# Autodesk Inventor assembly: 2024-210-Fixed-Shootaur
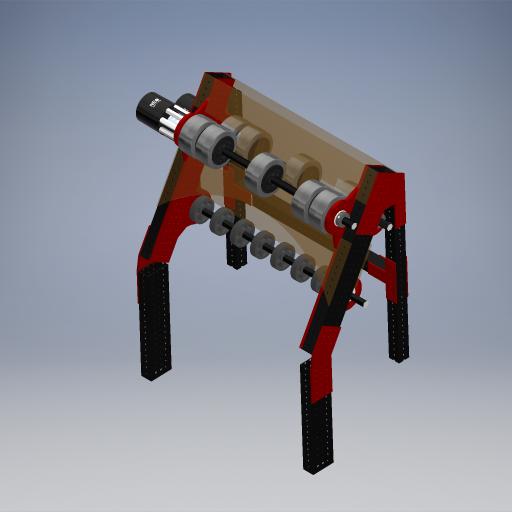
[picture p0: Inventor's stored thumbnail of the model, 512x512]
Saved by Autodesk Inventor 2024.2 (Build 282272000, 272)
## iProperties
Created: 2024-02-11
Part Number: 2024-210-Fixed-Shootaur
Document SubType Name: Assembly
Designer: rohan
Author: rohan
## Documents named in this file (23)
- C:\Users\rohan\OneDrive - Hillsborough County Public Schools\Robotics\FIRST-Robotics-Competition\Crescendo\Minotaur-Crescendo-Robot\Structure\Superstructure\Fixed Shooter\2024-210-Fixed-Shootaur.iam
- C:\Users\rohan\OneDrive - Hillsborough County Public Schools\Robotics\FIRST-Robotics-Competition\Crescendo\Minotaur-Crescendo-Robot\Structure\Superstructure\Fixed Shooter\2024-210-004-Back-Gusset.ipt
- C:\Users\rohan\OneDrive - Hillsborough County Public Schools\Robotics\FIRST-Robotics-Competition\Crescendo\Minotaur-Crescendo-Robot\Structure\Superstructure\Fixed Shooter\2024-210-005-Front-Gusset.ipt
- C:\Users\rohan\OneDrive - Hillsborough County Public Schools\Robotics\FIRST-Robotics-Competition\Crescendo\Minotaur-Crescendo-Robot\Structure\Superstructure\Fixed Shooter\2024-210-001-Shooter-Beam.ipt
- C:\Users\rohan\OneDrive - Hillsborough County Public Schools\Robotics\FIRST-Robotics-Competition\Crescendo\Minotaur-Crescendo-Robot\Structure\Superstructure\Fixed Shooter\2024-210-003-Front-Angle.ipt
- C:\Users\rohan\OneDrive - Hillsborough County Public Schools\Robotics\FIRST-Robotics-Competition\Crescendo\Minotaur-Crescendo-Robot\Structure\Superstructure\Fixed Shooter\2024-210-002-Backright-Support.ipt
- C:\Users\rohan\OneDrive - Hillsborough County Public Schools\Robotics\FIRST-Robotics-Competition\Crescendo\Minotaur-Crescendo-Robot\Structure\Superstructure\Fixed Shooter\2024-210-007-Left-Right-Support.ipt
- C:\Users\rohan\OneDrive - Hillsborough County Public Schools\Robotics\FIRST-Robotics-Competition\Crescendo\Minotaur-Crescendo-Robot\Structure\Gussets\THRIFYBOT-T-Gusset.ipt
- C:\Users\rohan\OneDrive - Hillsborough County Public Schools\Robotics\FIRST-Robotics-Competition\Crescendo\Minotaur-Crescendo-Robot\Structure\Superstructure\Polycarbonate-Note-Intakaur-Cover - Copy.ipt
- C:\Users\rohan\OneDrive - Hillsborough County Public Schools\Robotics\FIRST-Robotics-Competition\Crescendo\Minotaur-Crescendo-Robot\Structure\Superstructure\Fixed Shooter\2024-210-009-Shooter-Gusset-Plate.ipt
- C:\Users\rohan\OneDrive - Hillsborough County Public Schools\Robotics\FIRST-Robotics-Competition\Crescendo\Minotaur-Crescendo-Robot\Electronics\Neo-Brushless-Motors\NEO-Brushless-Motor-V1.1.ipt
- C:\Users\rohan\OneDrive - Hillsborough County Public Schools\Robotics\FIRST-Robotics-Competition\Crescendo\Minotaur-Crescendo-Robot\Motion\Adapters\0.5-inch-Hex-Shaft-Coupler.ipt
- C:\Users\rohan\OneDrive - Hillsborough County Public Schools\Robotics\FIRST-Robotics-Competition\Crescendo\Minotaur-Crescendo-Robot\Motion\Adapters\8mm-to-HEX.ipt
- C:\Users\rohan\OneDrive - Hillsborough County Public Schools\Robotics\FIRST-Robotics-Competition\Crescendo\Minotaur-Crescendo-Robot\Motion\Shafting\2024-210-010-Shooter-HEX-Shaft.ipt
- C:\Users\rohan\OneDrive - Hillsborough County Public Schools\Robotics\FIRST-Robotics-Competition\Crescendo\Minotaur-Crescendo-Robot\Motion\Wheels\3in-Colson-Performa.ipt
- C:\Users\rohan\OneDrive - Hillsborough County Public Schools\Robotics\FIRST-Robotics-Competition\Crescendo\Minotaur-Crescendo-Robot\Motion\Bearings\HEX-Bearing (1.125in OD).ipt
- C:\Users\rohan\OneDrive - Hillsborough County Public Schools\Robotics\FIRST-Robotics-Competition\Crescendo\Minotaur-Crescendo-Robot\Motion\Shafting\2024-210-011-Dead-Note-Guide.ipt
- C:\Users\rohan\OneDrive - Hillsborough County Public Schools\Robotics\FIRST-Robotics-Competition\Crescendo\Minotaur-Crescendo-Robot\Motion\Adapters\0.5-inch-HEX-Shaft-Collar (High Strength, Balanced).ipt
- C:\Users\rohan\OneDrive - Hillsborough County Public Schools\Robotics\FIRST-Robotics-Competition\Crescendo\Minotaur-Crescendo-Robot\Structure\Standoffs\Spacers__Standoffs.ipt
- C:\Users\rohan\OneDrive - Hillsborough County Public Schools\Robotics\FIRST-Robotics-Competition\Crescendo\Minotaur-Crescendo-Robot\Structure\Standoffs\Spacers__Standoffs\Aluminum Hex Standoff (No. 10x32 x 1.5Lg x 0.375OD).ipt
- C:\Users\rohan\OneDrive - Hillsborough County Public Schools\Robotics\FIRST-Robotics-Competition\Crescendo\Minotaur-Crescendo-Robot\Structure\Standoffs\Spacers__Standoffs\Aluminum Hex Standoff (No. 10x32 x 1.75Lg x 0.375OD).ipt
- C:\Users\rohan\OneDrive - Hillsborough County Public Schools\Robotics\FIRST-Robotics-Competition\Crescendo\Minotaur-Crescendo-Robot\Structure\Superstructure\Polycarbonate-Bottom-Shooter-Rest.ipt
- C:\Users\rohan\OneDrive - Hillsborough County Public Schools\Robotics\FIRST-Robotics-Competition\Crescendo\Minotaur-Crescendo-Robot\Motion\Wheels\2in-Compliant-Wheels-45A.ipt
## Components (63 placed, 21 different names)
1. 2024-210-004-Back-Gusset:1 — Flush:9, Mate:44, Flush:55, Flush:60
2. 2024-210-005-Front-Gusset:2 — Flush:23, Mate:22, Flush:24, Mate:25, Flush:26, Mate:26
3. 2024-210-001-Shooter-Beam:1 — Flush:23, Mate:22, Flush:24, Mate:38, Flush:48, Flush:49, Flush:52, Mate:40, Flush:53, Mate:44, Flush:55, Mate:169, Flush:57, Flush:58, Flush:60
4. 2024-210-002-Backright-Support:1 — Flush:9, Flush:19, Flush:20, Mate:13
5. 2024-210-004-Back-Gusset:4 — Flush:59
6. 2024-210-005-Front-Gusset:3 — Mate:21, Flush:21, Flush:22, Mate:23, Flush:25, Mate:24
7. 2024-210-001-Shooter-Beam:2 — Mate:21, Flush:21, Flush:22, Mate:39, Flush:50, Flush:51, Insert:8, Flush:59
8. 2024-210-002-Backright-Support:2 — Flush:19, Flush:20, Mate:13
9. 2024-210-003-Front-Angle:1 — Mate:25, Flush:26, Mate:26, Mate:28, Mate:36, Flush:44, Flush:54
10. 2024-210-003-Front-Angle:2 — Mate:23, Flush:25, Mate:24, Flush:29, Mate:35, Flush:43, Insert:7, Flush:54
11. 2024-210-007-Left-Right-Support:1 — Mate:28, Flush:29, Flush:42, Flush:45, Mate:43
12. THRIFYBOT-T-Gusset:1 — Flush:38, Flush:39, Mate:33, Mate:35, Flush:42, Flush:43, Insert:7
13. THRIFYBOT-T-Gusset:2 — Flush:38, Flush:39, Mate:33
14. THRIFYBOT-T-Gusset:3 — Mate:36, Flush:44, Flush:45
15. THRIFYBOT-T-Gusset:4 — Mate:43
16. Polycarbonate-Note-Intakaur-Cover - Copy:1 — Mate:38, Flush:48, Flush:49, Insert:8
17. 2024-210-009-Shooter-Gusset-Plate:1 — Mate:39, Flush:50, Flush:51, Symmetry:1, Mate:137, Mate:138, Mate:157, Mate:158, Mate:159, Mate:160
18. 2024-210-009-Shooter-Gusset-Plate:2 — Flush:52, Mate:40, Flush:53, Mate:58, Mate:59, Mate:67, Mate:68, Mate:95, Mate:103, Symmetry:1, Mate:135, Mate:136, Mate:147, Mate:148, Mate:150, Mate:151, Mate:152, Mate:153, Mate:155, Mate:156, Mate:161, Mate:162
19. NEO-Brushless-Motor-V1.1:1 — Mate:58, Mate:59, Mate:102, Mate:123, Mate:149
20. NEO-Brushless-Motor-V1.1:2 — Mate:67, Mate:68, Mate:94, Mate:122, Mate:154
21. 0.5-inch-Hex-Shaft-Coupler:1 — Mate:88, Mate:89, Mate:90, Mate:91, Mate:95, Mate:122
22. 8mm-to-HEX:1 — Mate:88, Mate:89, Mate:92, Mate:93, Mate:94
23. 2024-210-010-Shooter-HEX-Shaft:1 — Mate:90, Mate:91, Mate:92, Mate:116, Mate:117, Mate:118, Mate:119, Mate:124, Mate:125, Mate:126, Mate:127, Mate:131, Mate:132, Mate:163, Mate:164
24. 0.5-inch-Hex-Shaft-Coupler:5 — Mate:103, Mate:123
25. 8mm-to-HEX:5 — Mate:101, Mate:102
26. 2024-210-010-Shooter-HEX-Shaft:2 — Mate:104, Mate:105, Mate:106, Mate:107, Mate:110, Mate:111, Mate:112, Mate:113, Mate:129, Mate:130, Mate:166, Mate:167
27. 3in-Colson-Performa:1 — Mate:124, Mate:125, Mate:128, Mate:191
28. 3in-Colson-Performa:2 — Mate:110, Mate:111, Mate:114, Mate:189
29. 3in-Colson-Performa:3 — Mate:106, Mate:107, Mate:109, Mate:133
30. 3in-Colson-Performa:4 — Mate:104, Mate:105, Mate:109, Mate:192
31. 3in-Colson-Performa:5 — Mate:112, Mate:113, Mate:114
32. 3in-Colson-Performa:6 — Mate:116, Mate:117, Mate:120, Mate:190
33. 3in-Colson-Performa:7 — Mate:118, Mate:119, Mate:120
34. 3in-Colson-Performa:8 — Mate:126, Mate:127, Mate:128, Mate:134
35. 3in-Colson-Performa:9 — Mate:129, Mate:130, Mate:133
36. 3in-Colson-Performa:10 — Mate:131, Mate:132, Mate:134
37. HEX-Bearing (1.125in OD):1 — Mate:137, Mate:138, Mate:139, Mate:140
38. HEX-Bearing (1.125in OD):2 — Mate:135, Mate:136, Mate:188, Insert:9
39. 2024-210-011-Dead-Note-Guide:1 — Mate:139, Mate:140, Mate:188
40. Aluminum Hex Standoff (No. 10x32 x 1.5Lg x 0.375OD):6 — Mate:152, Mate:153
41. HEX-Bearing (1.125in OD):3 — Mate:155, Mate:156, Mate:192
42. HEX-Bearing (1.125in OD):4 — Mate:157, Mate:158, Mate:168, Mate:189
43. HEX-Bearing (1.125in OD):5 — Mate:161, Mate:162, Mate:191
44. HEX-Bearing (1.125in OD):6 — Mate:159, Mate:160, Mate:165, Mate:190
45. 0.5-inch-HEX-Shaft-Collar (High Strength, Balanced):5 — Mate:163, Mate:164, Mate:165
46. 0.5-inch-HEX-Shaft-Collar (High Strength, Balanced):7 — Mate:166, Mate:167, Mate:168
47. Polycarbonate-Bottom-Shooter-Rest:1 — Mate:169, Flush:57, Flush:58
48. Aluminum Hex Standoff (No. 10x32 x 1.75Lg x 0.375OD):1 — Mate:147, Mate:148
49. Aluminum Hex Standoff (No. 10x32 x 1.75Lg x 0.375OD):7
50. Aluminum Hex Standoff (No. 10x32 x 1.75Lg x 0.375OD):8
51. Aluminum Hex Standoff (No. 10x32 x 1.75Lg x 0.375OD):9
52. Aluminum Hex Standoff (No. 10x32 x 1.75Lg x 0.375OD):10
53. Aluminum Hex Standoff (No. 10x32 x 1.75Lg x 0.375OD):11 — Mate:149
54. Aluminum Hex Standoff (No. 10x32 x 1.75Lg x 0.375OD):4 — Mate:150, Mate:151
55. Aluminum Hex Standoff (No. 10x32 x 1.75Lg x 0.375OD):12 — Mate:154
56. 2in-Compliant-Wheels-45A:8 — Insert:9
57. 2in-Compliant-Wheels-45A:9
58. 2in-Compliant-Wheels-45A:10
59. 2in-Compliant-Wheels-45A:11
60. 2in-Compliant-Wheels-45A:12
61. 2in-Compliant-Wheels-45A:13
62. 2in-Compliant-Wheels-45A:14
63. 2in-Compliant-Wheels-45A:15
## Component patterns: (6 elements, first: Aluminum Hex Standoff (No. 10x32 x 1.75Lg x 0.375OD):1), (2 elements, first: Aluminum Hex Standoff (No. 10x32 x 1.75Lg x 0.375OD):4), (8 elements, first: 2in-Compliant-Wheels-45A:8)
## Relationships (138: Mate 101, Flush 31, Insert 5, Symmetry 1)
- Flush:9: 2024-210-004-Back-Gusset:1 ↔ 2024-210-002-Backright-Support:1
- [Mate]: 2024-210-004-Back-Gusset:4 ↔ 2024-210-001-Shooter-Beam:2
- [Flush]: 2024-210-004-Back-Gusset:4 ↔ 2024-210-001-Shooter-Beam:2
- [Insert]: 2024-210-004-Back-Gusset:4 ↔ 2024-210-001-Shooter-Beam:2
- [Mate]: 2024-210-004-Back-Gusset:4 ↔ 2024-210-002-Backright-Support:2
- [Insert]: 2024-210-004-Back-Gusset:4 ↔ 2024-210-002-Backright-Support:2
- Flush:19: 2024-210-002-Backright-Support:1 ↔ 2024-210-002-Backright-Support:2
- Flush:20: 2024-210-002-Backright-Support:1 ↔ 2024-210-002-Backright-Support:2
- Mate:13 (381 mm): 2024-210-002-Backright-Support:1 ↔ 2024-210-002-Backright-Support:2
- Mate:21: 2024-210-005-Front-Gusset:3 ↔ 2024-210-001-Shooter-Beam:2
- Flush:21: 2024-210-005-Front-Gusset:3 ↔ 2024-210-001-Shooter-Beam:2
- Flush:22: 2024-210-005-Front-Gusset:3 ↔ 2024-210-001-Shooter-Beam:2
- Flush:23: 2024-210-005-Front-Gusset:2 ↔ 2024-210-001-Shooter-Beam:1
- Mate:22: 2024-210-005-Front-Gusset:2 ↔ 2024-210-001-Shooter-Beam:1
- Flush:24: 2024-210-005-Front-Gusset:2 ↔ 2024-210-001-Shooter-Beam:1
- Mate:23: 2024-210-005-Front-Gusset:3 ↔ 2024-210-003-Front-Angle:2
- Flush:25: 2024-210-005-Front-Gusset:3 ↔ 2024-210-003-Front-Angle:2
- Mate:24: 2024-210-005-Front-Gusset:3 ↔ 2024-210-003-Front-Angle:2
- Mate:25: 2024-210-005-Front-Gusset:2 ↔ 2024-210-003-Front-Angle:1
- Flush:26: 2024-210-005-Front-Gusset:2 ↔ 2024-210-003-Front-Angle:1
- Mate:26: 2024-210-005-Front-Gusset:2 ↔ 2024-210-003-Front-Angle:1
- Mate:28: 2024-210-003-Front-Angle:1 ↔ 2024-210-007-Left-Right-Support:1
- Flush:29: 2024-210-003-Front-Angle:2 ↔ 2024-210-007-Left-Right-Support:1
- Flush:38: THRIFYBOT-T-Gusset:1 ↔ THRIFYBOT-T-Gusset:2
- Flush:39: THRIFYBOT-T-Gusset:1 ↔ THRIFYBOT-T-Gusset:2
- Mate:33 (25.4 mm): THRIFYBOT-T-Gusset:1 ↔ THRIFYBOT-T-Gusset:2
- [Flush]: THRIFYBOT-T-Gusset:3 ↔ THRIFYBOT-T-Gusset:4
- [Flush]: THRIFYBOT-T-Gusset:3 ↔ THRIFYBOT-T-Gusset:4
- [Mate] (25.4 mm): THRIFYBOT-T-Gusset:3 ↔ THRIFYBOT-T-Gusset:4
- Mate:35: 2024-210-003-Front-Angle:2 ↔ THRIFYBOT-T-Gusset:1
- Flush:42: 2024-210-007-Left-Right-Support:1 ↔ THRIFYBOT-T-Gusset:1
- Flush:43: 2024-210-003-Front-Angle:2 ↔ THRIFYBOT-T-Gusset:1
- Mate:36: 2024-210-003-Front-Angle:1 ↔ THRIFYBOT-T-Gusset:3
- Flush:44: 2024-210-003-Front-Angle:1 ↔ THRIFYBOT-T-Gusset:3
- Flush:45: 2024-210-007-Left-Right-Support:1 ↔ THRIFYBOT-T-Gusset:3
- Mate:38: 2024-210-001-Shooter-Beam:1 ↔ Polycarbonate-Note-Intakaur-Cover - Copy:1
- Flush:48: 2024-210-001-Shooter-Beam:1 ↔ Polycarbonate-Note-Intakaur-Cover - Copy:1
- Flush:49: 2024-210-001-Shooter-Beam:1 ↔ Polycarbonate-Note-Intakaur-Cover - Copy:1
- Insert:7: 2024-210-003-Front-Angle:2 ↔ THRIFYBOT-T-Gusset:1
- Mate:39: 2024-210-001-Shooter-Beam:2 ↔ 2024-210-009-Shooter-Gusset-Plate:1
- Flush:50: 2024-210-001-Shooter-Beam:2 ↔ 2024-210-009-Shooter-Gusset-Plate:1
- Flush:51: 2024-210-001-Shooter-Beam:2 ↔ 2024-210-009-Shooter-Gusset-Plate:1
- Flush:52: 2024-210-001-Shooter-Beam:1 ↔ 2024-210-009-Shooter-Gusset-Plate:2
- Mate:40: 2024-210-001-Shooter-Beam:1 ↔ 2024-210-009-Shooter-Gusset-Plate:2
- Flush:53: 2024-210-001-Shooter-Beam:1 ↔ 2024-210-009-Shooter-Gusset-Plate:2
- Mate:43: 2024-210-007-Left-Right-Support:1 ↔ THRIFYBOT-T-Gusset:4
- Mate:44: 2024-210-004-Back-Gusset:1 ↔ 2024-210-001-Shooter-Beam:1
- Flush:54: 2024-210-003-Front-Angle:1 ↔ 2024-210-003-Front-Angle:2
- Insert:8: 2024-210-001-Shooter-Beam:2 ↔ Polycarbonate-Note-Intakaur-Cover - Copy:1
- Mate:58: 2024-210-009-Shooter-Gusset-Plate:2 ↔ NEO-Brushless-Motor-V1.1:1
- Mate:59: 2024-210-009-Shooter-Gusset-Plate:2 ↔ NEO-Brushless-Motor-V1.1:1
- Mate:67: 2024-210-009-Shooter-Gusset-Plate:2 ↔ NEO-Brushless-Motor-V1.1:2
- Mate:68: 2024-210-009-Shooter-Gusset-Plate:2 ↔ NEO-Brushless-Motor-V1.1:2
- Flush:55: 2024-210-004-Back-Gusset:1 ↔ 2024-210-001-Shooter-Beam:1
- Mate:88: 0.5-inch-Hex-Shaft-Coupler:1 ↔ 8mm-to-HEX:1
- Mate:89: 0.5-inch-Hex-Shaft-Coupler:1 ↔ 8mm-to-HEX:1
- Mate:90: 0.5-inch-Hex-Shaft-Coupler:1 ↔ 2024-210-010-Shooter-HEX-Shaft:1
- Mate:91: 0.5-inch-Hex-Shaft-Coupler:1 ↔ 2024-210-010-Shooter-HEX-Shaft:1
- Mate:92: 8mm-to-HEX:1 ↔ 2024-210-010-Shooter-HEX-Shaft:1
- Mate:93: 8mm-to-HEX:1
- Mate:94: NEO-Brushless-Motor-V1.1:2 ↔ 8mm-to-HEX:1
- Mate:95: 2024-210-009-Shooter-Gusset-Plate:2 ↔ 0.5-inch-Hex-Shaft-Coupler:1
- [Mate]: 0.5-inch-Hex-Shaft-Coupler:5 ↔ 8mm-to-HEX:5
- [Mate]: 0.5-inch-Hex-Shaft-Coupler:5 ↔ 8mm-to-HEX:5
- [Mate]: 0.5-inch-Hex-Shaft-Coupler:5 ↔ 2024-210-010-Shooter-HEX-Shaft:2
- [Mate]: 0.5-inch-Hex-Shaft-Coupler:5 ↔ 2024-210-010-Shooter-HEX-Shaft:2
- [Mate]: 8mm-to-HEX:5 ↔ 2024-210-010-Shooter-HEX-Shaft:2
- Mate:101: 8mm-to-HEX:5
- Mate:102: NEO-Brushless-Motor-V1.1:1 ↔ 8mm-to-HEX:5
- Mate:103: 2024-210-009-Shooter-Gusset-Plate:2 ↔ 0.5-inch-Hex-Shaft-Coupler:5
- Mate:104: 2024-210-010-Shooter-HEX-Shaft:2 ↔ 3in-Colson-Performa:4
- Mate:105: 2024-210-010-Shooter-HEX-Shaft:2 ↔ 3in-Colson-Performa:4
- Mate:106: 2024-210-010-Shooter-HEX-Shaft:2 ↔ 3in-Colson-Performa:3
- Mate:107: 2024-210-010-Shooter-HEX-Shaft:2 ↔ 3in-Colson-Performa:3
- Mate:109: 3in-Colson-Performa:3 ↔ 3in-Colson-Performa:4
- Mate:110: 2024-210-010-Shooter-HEX-Shaft:2 ↔ 3in-Colson-Performa:2
- Mate:111: 2024-210-010-Shooter-HEX-Shaft:2 ↔ 3in-Colson-Performa:2
- Mate:112: 2024-210-010-Shooter-HEX-Shaft:2 ↔ 3in-Colson-Performa:5
- Mate:113: 2024-210-010-Shooter-HEX-Shaft:2 ↔ 3in-Colson-Performa:5
- Mate:114: 3in-Colson-Performa:2 ↔ 3in-Colson-Performa:5
- Mate:116: 2024-210-010-Shooter-HEX-Shaft:1 ↔ 3in-Colson-Performa:6
- Mate:117: 2024-210-010-Shooter-HEX-Shaft:1 ↔ 3in-Colson-Performa:6
- Mate:118: 2024-210-010-Shooter-HEX-Shaft:1 ↔ 3in-Colson-Performa:7
- Mate:119: 2024-210-010-Shooter-HEX-Shaft:1 ↔ 3in-Colson-Performa:7
- Mate:120: 3in-Colson-Performa:6 ↔ 3in-Colson-Performa:7
- Mate:122: NEO-Brushless-Motor-V1.1:2 ↔ 0.5-inch-Hex-Shaft-Coupler:1
- Mate:123: NEO-Brushless-Motor-V1.1:1 ↔ 0.5-inch-Hex-Shaft-Coupler:5
- Mate:124: 2024-210-010-Shooter-HEX-Shaft:1 ↔ 3in-Colson-Performa:1
- Mate:125: 2024-210-010-Shooter-HEX-Shaft:1 ↔ 3in-Colson-Performa:1
- Mate:126: 2024-210-010-Shooter-HEX-Shaft:1 ↔ 3in-Colson-Performa:8
- Mate:127: 2024-210-010-Shooter-HEX-Shaft:1 ↔ 3in-Colson-Performa:8
- Mate:128: 3in-Colson-Performa:1 ↔ 3in-Colson-Performa:8
- Mate:129: 2024-210-010-Shooter-HEX-Shaft:2 ↔ 3in-Colson-Performa:9
- Mate:130: 2024-210-010-Shooter-HEX-Shaft:2 ↔ 3in-Colson-Performa:9
- Mate:131: 2024-210-010-Shooter-HEX-Shaft:1 ↔ 3in-Colson-Performa:10
- Mate:132: 2024-210-010-Shooter-HEX-Shaft:1 ↔ 3in-Colson-Performa:10
- Symmetry:1: 2024-210-009-Shooter-Gusset-Plate:1 ↔ 2024-210-009-Shooter-Gusset-Plate:2
- Mate:133 (81.28 mm): 3in-Colson-Performa:3 ↔ 3in-Colson-Performa:9
- Mate:134 (81.28 mm): 3in-Colson-Performa:8 ↔ 3in-Colson-Performa:10
- Mate:135: 2024-210-009-Shooter-Gusset-Plate:2 ↔ HEX-Bearing (1.125in OD):2
- Mate:136: 2024-210-009-Shooter-Gusset-Plate:2 ↔ HEX-Bearing (1.125in OD):2
- Mate:137: 2024-210-009-Shooter-Gusset-Plate:1 ↔ HEX-Bearing (1.125in OD):1
- Mate:138: 2024-210-009-Shooter-Gusset-Plate:1 ↔ HEX-Bearing (1.125in OD):1
- Mate:139: HEX-Bearing (1.125in OD):1 ↔ 2024-210-011-Dead-Note-Guide:1
- Mate:140: HEX-Bearing (1.125in OD):1 ↔ 2024-210-011-Dead-Note-Guide:1
- Mate:147: 2024-210-009-Shooter-Gusset-Plate:2 ↔ Aluminum Hex Standoff (No. 10x32 x 1.75Lg x 0.375OD):1
- Mate:148: 2024-210-009-Shooter-Gusset-Plate:2 ↔ Aluminum Hex Standoff (No. 10x32 x 1.75Lg x 0.375OD):1
- Mate:149: NEO-Brushless-Motor-V1.1:1 ↔ Aluminum Hex Standoff (No. 10x32 x 1.75Lg x 0.375OD):11
- Mate:150: 2024-210-009-Shooter-Gusset-Plate:2 ↔ Aluminum Hex Standoff (No. 10x32 x 1.75Lg x 0.375OD):4
- Mate:151: 2024-210-009-Shooter-Gusset-Plate:2 ↔ Aluminum Hex Standoff (No. 10x32 x 1.75Lg x 0.375OD):4
- Mate:152: 2024-210-009-Shooter-Gusset-Plate:2 ↔ Aluminum Hex Standoff (No. 10x32 x 1.5Lg x 0.375OD):6
- Mate:153: 2024-210-009-Shooter-Gusset-Plate:2 ↔ Aluminum Hex Standoff (No. 10x32 x 1.5Lg x 0.375OD):6
- Mate:154: NEO-Brushless-Motor-V1.1:2 ↔ Aluminum Hex Standoff (No. 10x32 x 1.75Lg x 0.375OD):12
- Mate:155: 2024-210-009-Shooter-Gusset-Plate:2 ↔ HEX-Bearing (1.125in OD):3
- Mate:156: 2024-210-009-Shooter-Gusset-Plate:2 ↔ HEX-Bearing (1.125in OD):3
- Mate:157: 2024-210-009-Shooter-Gusset-Plate:1 ↔ HEX-Bearing (1.125in OD):4
- Mate:158: 2024-210-009-Shooter-Gusset-Plate:1 ↔ HEX-Bearing (1.125in OD):4
- Mate:159: 2024-210-009-Shooter-Gusset-Plate:1 ↔ HEX-Bearing (1.125in OD):6
- Mate:160: 2024-210-009-Shooter-Gusset-Plate:1 ↔ HEX-Bearing (1.125in OD):6
- Mate:161: 2024-210-009-Shooter-Gusset-Plate:2 ↔ HEX-Bearing (1.125in OD):5
- Mate:162: 2024-210-009-Shooter-Gusset-Plate:2 ↔ HEX-Bearing (1.125in OD):5
- Mate:163: 2024-210-010-Shooter-HEX-Shaft:1 ↔ 0.5-inch-HEX-Shaft-Collar (High Strength, Balanced):5
- Mate:164: 2024-210-010-Shooter-HEX-Shaft:1 ↔ 0.5-inch-HEX-Shaft-Collar (High Strength, Balanced):5
- Mate:165: HEX-Bearing (1.125in OD):6 ↔ 0.5-inch-HEX-Shaft-Collar (High Strength, Balanced):5
- Mate:166: 2024-210-010-Shooter-HEX-Shaft:2 ↔ 0.5-inch-HEX-Shaft-Collar (High Strength, Balanced):7
- Mate:167: 2024-210-010-Shooter-HEX-Shaft:2 ↔ 0.5-inch-HEX-Shaft-Collar (High Strength, Balanced):7
- Mate:168: HEX-Bearing (1.125in OD):4 ↔ 0.5-inch-HEX-Shaft-Collar (High Strength, Balanced):7
- Mate:169: 2024-210-001-Shooter-Beam:1 ↔ Polycarbonate-Bottom-Shooter-Rest:1
- Flush:57: 2024-210-001-Shooter-Beam:1 ↔ Polycarbonate-Bottom-Shooter-Rest:1
- Flush:58: 2024-210-001-Shooter-Beam:1 ↔ Polycarbonate-Bottom-Shooter-Rest:1
- Mate:188: HEX-Bearing (1.125in OD):2 ↔ 2024-210-011-Dead-Note-Guide:1
- Mate:189: 3in-Colson-Performa:2 ↔ HEX-Bearing (1.125in OD):4
- Mate:190: 3in-Colson-Performa:6 ↔ HEX-Bearing (1.125in OD):6
- Mate:191: 3in-Colson-Performa:1 ↔ HEX-Bearing (1.125in OD):5
- Mate:192: 3in-Colson-Performa:4 ↔ HEX-Bearing (1.125in OD):3
- Flush:59: 2024-210-004-Back-Gusset:4 ↔ 2024-210-001-Shooter-Beam:2
- Flush:60: 2024-210-004-Back-Gusset:1 ↔ 2024-210-001-Shooter-Beam:1
- Insert:9 (-13.3096 mm): HEX-Bearing (1.125in OD):2 ↔ 2in-Compliant-Wheels-45A:8
## Named parameters: d24_d6 = 0 mm, d25_d7 = 0 mm, d26_d8 = 0 mm, d33_d15 = 0 mm, d35_d17 = 0 mm, d89_d86 = 0 mm, d90_d87 = 0 mm, d91_d88 = 25.4 mm, d178_d169 = 0 mm, d179_d170 = 0 mm, d180_d171 = 0 mm, d181_d172 = 0 mm, d182_d173 = 0 mm
